# Autodesk Inventor assembly: switch_assembly
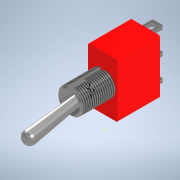
[picture p0: Inventor's stored thumbnail of the model, 180x180]
Saved by Autodesk Inventor 2022.2 (Build 262287000, 287)
## iProperties
Created: 2022-01-24
Part Number: switch_assembly
Document SubType Name: Assembly
Designer: hugof
Author: hugof
## Documents named in this file (3)
- C:\Users\hugof\Documents\GitHub\tco-cad\switch_mount\switch_assembly.iam
- C:\Users\hugof\Documents\GitHub\tco-cad\switch_mount\switch_case.ipt
- C:\Users\hugof\Documents\GitHub\tco-cad\switch_mount\switch_stem.ipt
## Components (2 placed, 2 different names)
1. switch_case:1 — Mate:1, Angle:1
2. switch_stem:1 — Mate:1, Angle:1
## Relationships (2: Mate 1, Angle 1)
- Mate:1 (1 mm): switch_case:1 ↔ switch_stem:1
- Angle:1 (10 deg): switch_case:1 ↔ switch_stem:1
